# Autodesk Inventor assembly: 組合2
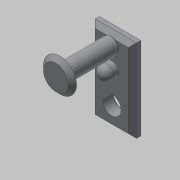
[picture p0: Inventor's stored thumbnail of the model, 180x180]
Saved by Autodesk Inventor 2018 (Build 220112000, 112)
## iProperties
Created: 2020-09-19
Part Number: 組合2
Material: 一般
Document SubType Name: Assembly
Designer: 王鼎鈞
Author: 王鼎鈞
## Documents named in this file (4)
- D:\2020嚴家明 功課黨\組合2.iam
- D:\2020嚴家明 功課黨\exercise2-1.ipt
- D:\2020嚴家明 功課黨\exercise2-2.ipt
- D:\2020嚴家明 功課黨\exercise2-3.ipt
## Components (3 placed, 3 different names)
1. exercise2-1:1 — 貼合:1, 貼合:2, 插入:1
2. exercise2-2:1 — 插入:1
3. exercise2-3:1 — 貼合:1, 貼合:2
## Relationships (3: Mate 2, Insert 1)
- 貼合:1 [Mate]: exercise2-1:1 ↔ exercise2-3:1
- 貼合:2 [Mate]: exercise2-1:1 ↔ exercise2-3:1
- 插入:1 [Insert]: exercise2-1:1 ↔ exercise2-2:1
